# Autodesk Inventor assembly: Elevator
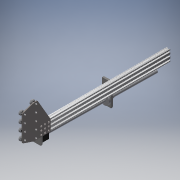
[picture p0: Inventor's stored thumbnail of the model, 180x180]
Saved by Autodesk Inventor 2017 (Build 210142000, 142)
## iProperties
Created: 2016-12-12
Part Number: Elevator
Document SubType Name: Assembly
Designer: umr
Author: umr
## Documents named in this file (12)
- D:\SeniorProject\Models2\Elevator.iam
- D:\SeniorProject\Models2\Gantry Plate.ipt
- D:\SeniorProject\Models2\M5 Screw with Tee Nut.iam
- D:\SeniorProject\Models2\Solid Wheel with Eccentric Spacer Assembly.iam
- D:\SeniorProject\Models2\L_Fixer.ipt
- D:\SeniorProject\Models2\DriverElevatorConnection.ipt
- D:\SeniorProject\Models2\L_Fixer2.ipt
- D:\SeniorProject\Models2\ScrewDriver.ipt
- D:\SeniorProject\Models2\PowerScrewNut.ipt
- D:\SeniorProject\Models2\MotorFixer.ipt
- D:\SeniorProject\Models2\Elevator Track.ipt
- D:\SeniorProject\Models2\Motor.ipt
## Components (32 placed, 11 different names)
1. Gantry Plate:1 — Mate:1, Mate:2, Mate:3, Mate:4, Mate:5, Mate:6, Mate:7, Mate:8, Mate:9, Mate:11, Mate:12, Mate:13, Mate:14, Mate:16, Mate:17, Mate:18, Mate:21, Mate:22, Mate:26, Mate:27, Mate:28, Mate:29, Mate:30, Mate:31, Mate:32, Mate:33, Mate:34, Mate:35, Mate:36, Mate:37, Mate:38, Mate:39, Mate:40, Mate:41, Mate:42, Mate:43
2. M5 Screw with Tee Nut:1 [sub-assembly] — Mate:1, Mate:2
3. M5 Screw with Tee Nut:2 [sub-assembly] — Mate:3, Mate:14
4. M5 Screw with Tee Nut:3 [sub-assembly] — Mate:4, Mate:11
5. M5 Screw with Tee Nut:4 [sub-assembly] — Mate:5, Mate:18
6. M5 Screw with Tee Nut:5 [sub-assembly] — Mate:6, Mate:12
7. M5 Screw with Tee Nut:6 [sub-assembly] — Mate:7, Mate:13, Mate:56, Mate:57
8. M5 Screw with Tee Nut:7 [sub-assembly] — Mate:8, Mate:16
9. M5 Screw with Tee Nut:8 [sub-assembly] — Mate:9, Mate:17, Mate:58
10. M5 Screw with Tee Nut:9 [sub-assembly] — Mate:21, Mate:22
11. Solid Wheel with Eccentric Spacer Assembly:1 [sub-assembly] — Mate:29, Mate:43
12. Solid Wheel with Eccentric Spacer Assembly:2 [sub-assembly] — Mate:26, Mate:40
13. Solid Wheel with Eccentric Spacer Assembly:3 [sub-assembly] — Mate:27, Mate:39
14. Solid Wheel with Eccentric Spacer Assembly:4 [sub-assembly] — Mate:28, Mate:41
15. Solid Wheel with Eccentric Spacer Assembly:5 [sub-assembly] — Mate:30, Mate:42
16. Solid Wheel with Eccentric Spacer Assembly:6 [sub-assembly] — Mate:31, Mate:35
17. Solid Wheel with Eccentric Spacer Assembly:7 [sub-assembly] — Mate:32, Mate:36
18. Solid Wheel with Eccentric Spacer Assembly:8 [sub-assembly] — Mate:33, Mate:37
19. Solid Wheel with Eccentric Spacer Assembly:10 [sub-assembly] — Mate:34, Mate:38
20. L_Fixer:1 — Mate:44, Mate:45, Mate:46, Mate:47, Mate:48, Mate:49, Mate:69, Mate:70, Mate:71
21. M5 Screw with Tee Nut:10 [sub-assembly] — Mate:44, Mate:47, Mate:67
22. M5 Screw with Tee Nut:11 [sub-assembly] — Mate:45, Mate:48, Mate:68
23. M5 Screw with Tee Nut:12 [sub-assembly] — Mate:46, Mate:49, Mate:66
24. DriverElevatorConnection:1 — Mate:50, Mate:51, Mate:52, Mate:53, Mate:55
25. L_Fixer2:1 — Mate:50, Mate:51, Mate:52, Mate:59, Mate:60, Mate:61, Mate:62
26. ScrewDriver:1 — Mate:53, Mate:54, Mate:72, Mate:73
27. PowerScrewNut:1 — Mate:54, Mate:55
28. MotorFixer:1 — Mate:69, Mate:70, Mate:71, Mate:74
29. Elevator Track:1 — Mate:56, Mate:57, Mate:58, Mate:63, Mate:64, Mate:65, Mate:66, Mate:67, Mate:68
30. M5 Screw with Tee Nut:13 [sub-assembly] — Mate:59, Mate:62, Mate:63, Mate:64
31. M5 Screw with Tee Nut:14 [sub-assembly] — Mate:60, Mate:61, Mate:65
32. Motor:1 — Mate:72, Mate:73, Mate:74
## Relationships (67: Mate 67)
- Mate:1: Gantry Plate:1 ↔ M5 Screw with Tee Nut:1
- Mate:2: Gantry Plate:1 ↔ M5 Screw with Tee Nut:1
- Mate:3: Gantry Plate:1 ↔ M5 Screw with Tee Nut:2
- Mate:4: Gantry Plate:1 ↔ M5 Screw with Tee Nut:3
- Mate:5: Gantry Plate:1 ↔ M5 Screw with Tee Nut:4
- Mate:6: Gantry Plate:1 ↔ M5 Screw with Tee Nut:5
- Mate:7: Gantry Plate:1 ↔ M5 Screw with Tee Nut:6
- Mate:8: Gantry Plate:1 ↔ M5 Screw with Tee Nut:7
- Mate:9: Gantry Plate:1 ↔ M5 Screw with Tee Nut:8
- Mate:11: Gantry Plate:1 ↔ M5 Screw with Tee Nut:3
- Mate:12: Gantry Plate:1 ↔ M5 Screw with Tee Nut:5
- Mate:13: Gantry Plate:1 ↔ M5 Screw with Tee Nut:6
- Mate:14: Gantry Plate:1 ↔ M5 Screw with Tee Nut:2
- Mate:16: Gantry Plate:1 ↔ M5 Screw with Tee Nut:7
- Mate:17: Gantry Plate:1 ↔ M5 Screw with Tee Nut:8
- Mate:18: Gantry Plate:1 ↔ M5 Screw with Tee Nut:4
- Mate:21: Gantry Plate:1 ↔ M5 Screw with Tee Nut:9
- Mate:22: Gantry Plate:1 ↔ M5 Screw with Tee Nut:9
- Mate:26: Gantry Plate:1 ↔ Solid Wheel with Eccentric Spacer Assembly:2
- Mate:27: Gantry Plate:1 ↔ Solid Wheel with Eccentric Spacer Assembly:3
- Mate:28: Gantry Plate:1 ↔ Solid Wheel with Eccentric Spacer Assembly:4
- Mate:29: Gantry Plate:1 ↔ Solid Wheel with Eccentric Spacer Assembly:1
- Mate:30: Gantry Plate:1 ↔ Solid Wheel with Eccentric Spacer Assembly:5
- Mate:31: Gantry Plate:1 ↔ Solid Wheel with Eccentric Spacer Assembly:6
- Mate:32: Gantry Plate:1 ↔ Solid Wheel with Eccentric Spacer Assembly:7
- Mate:33: Gantry Plate:1 ↔ Solid Wheel with Eccentric Spacer Assembly:8
- Mate:34: Gantry Plate:1 ↔ Solid Wheel with Eccentric Spacer Assembly:10
- Mate:35: Gantry Plate:1 ↔ Solid Wheel with Eccentric Spacer Assembly:6
- Mate:36: Gantry Plate:1 ↔ Solid Wheel with Eccentric Spacer Assembly:7
- Mate:37: Gantry Plate:1 ↔ Solid Wheel with Eccentric Spacer Assembly:8
- Mate:38: Gantry Plate:1 ↔ Solid Wheel with Eccentric Spacer Assembly:10
- Mate:39: Gantry Plate:1 ↔ Solid Wheel with Eccentric Spacer Assembly:3
- Mate:40: Gantry Plate:1 ↔ Solid Wheel with Eccentric Spacer Assembly:2
- Mate:41: Gantry Plate:1 ↔ Solid Wheel with Eccentric Spacer Assembly:4
- Mate:42: Gantry Plate:1 ↔ Solid Wheel with Eccentric Spacer Assembly:5
- Mate:43: Gantry Plate:1 ↔ Solid Wheel with Eccentric Spacer Assembly:1
- Mate:44: L_Fixer:1 ↔ M5 Screw with Tee Nut:10
- Mate:45: L_Fixer:1 ↔ M5 Screw with Tee Nut:11
- Mate:46: L_Fixer:1 ↔ M5 Screw with Tee Nut:12
- Mate:47: L_Fixer:1 ↔ M5 Screw with Tee Nut:10
- Mate:48: L_Fixer:1 ↔ M5 Screw with Tee Nut:11
- Mate:49: L_Fixer:1 ↔ M5 Screw with Tee Nut:12
- Mate:50: DriverElevatorConnection:1 ↔ L_Fixer2:1
- Mate:51: DriverElevatorConnection:1 ↔ L_Fixer2:1
- Mate:52: DriverElevatorConnection:1 ↔ L_Fixer2:1
- Mate:53: DriverElevatorConnection:1 ↔ ScrewDriver:1
- Mate:54: ScrewDriver:1 ↔ PowerScrewNut:1
- Mate:55: DriverElevatorConnection:1 ↔ PowerScrewNut:1
- Mate:56: M5 Screw with Tee Nut:6 ↔ Elevator Track:1
- Mate:57: M5 Screw with Tee Nut:6 ↔ Elevator Track:1
- Mate:58: M5 Screw with Tee Nut:8 ↔ Elevator Track:1
- Mate:59: L_Fixer2:1 ↔ M5 Screw with Tee Nut:13
- Mate:60: L_Fixer2:1 ↔ M5 Screw with Tee Nut:14
- Mate:61: L_Fixer2:1 ↔ M5 Screw with Tee Nut:14
- Mate:62: L_Fixer2:1 ↔ M5 Screw with Tee Nut:13
- Mate:63: Elevator Track:1 ↔ M5 Screw with Tee Nut:13
- Mate:64: Elevator Track:1 ↔ M5 Screw with Tee Nut:13
- Mate:65: Elevator Track:1 ↔ M5 Screw with Tee Nut:14
- Mate:66: M5 Screw with Tee Nut:12 ↔ Elevator Track:1
- Mate:67: M5 Screw with Tee Nut:10 ↔ Elevator Track:1
- Mate:68: M5 Screw with Tee Nut:11 ↔ Elevator Track:1
- Mate:69: L_Fixer:1 ↔ MotorFixer:1
- Mate:70: L_Fixer:1 ↔ MotorFixer:1
- Mate:71: L_Fixer:1 ↔ MotorFixer:1
- Mate:72: ScrewDriver:1 ↔ Motor:1
- Mate:73: ScrewDriver:1 ↔ Motor:1
- Mate:74: MotorFixer:1 ↔ Motor:1
